# Autodesk Inventor assembly: приводной валь
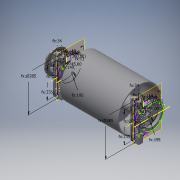
[picture p0: Inventor's stored thumbnail of the model, 180x180]
Saved by Autodesk Inventor 2018.3 (Build 223284000, 284)
## iProperties
Created: 2018-05-10
Part Number: приводной валь
Material: Типовые
Document SubType Name: Assembly
Designer: kriku
Mass: 17391.3 g
Surface Area: 20333.4 cm^2
Volume: 13778.9 cm^3
Density: 1.26217 g/cm^3
Author: kriku
## Documents named in this file (6)
- C:\Users\kriku\OneDrive\Рабочий стол\6 семестр\курсач ДМ\deadmash\Куча инви\приводной валь.iam
- C:\Users\kriku\OneDrive\Рабочий стол\6 семестр\курсач ДМ\deadmash\Куча инви\корпус подшипника1.ipt
- C:\Users\kriku\Downloads\barabashka.ipt
- C:\Users\kriku\Downloads\privodnoi_val.ipt
- C:\Users\kriku\OneDrive\Документы\Inventor\Content Center Files\R2018\ru-RU\Bearing 1000 GOST 28428-90\Подшипник 1214 ГОСТ 28428-90.ipt
- C:\Users\kriku\OneDrive\Документы\Inventor\Content Center Files\R2018\ru-RU\End Cap GOST 13219·10-81\Крышка торцовая МВ 125x70 ГОСТ 13219.10-81.ipt
## Components (7 placed, 5 different names)
1. корпус подшипника1:1 — Угол:1, Совмещение:6, Заподлицо:3
2. корпус подшипника1:2 — Угол:2, Совмещение:5, Заподлицо:2
3. barabashka:1 — Цилиндрический:1, Заподлицо:1
4. privodnoi_val:1 — Цилиндрический:1, Заподлицо:1, Совмещение:1, Совмещение:2, Совмещение:3, Совмещение:4, Совмещение:5, Совмещение:6, Совмещение:7
5. Подшипник 1000 ГОСТ 28428-90 1214:1 — Совмещение:1, Совмещение:2, Заподлицо:2
6. Подшипник 1000 ГОСТ 28428-90 1214:2 — Совмещение:3, Совмещение:4, Заподлицо:3
7. Крышка торцовая ГОСТ 13219.10-81 МВ 125x70:1 — Совмещение:7
## Relationships (13: Mate 7, Flush 3, Angle 2, CylindricalJoint 1)
- Цилиндрический:1 [CylindricalJoint]: barabashka:1 ↔ privodnoi_val:1
- Заподлицо:1 [Flush]: barabashka:1 ↔ privodnoi_val:1
- Совмещение:1 [Mate]: privodnoi_val:1 ↔ Подшипник 1000 ГОСТ 28428-90 1214:1
- Совмещение:2 [Mate]: privodnoi_val:1 ↔ Подшипник 1000 ГОСТ 28428-90 1214:1
- Совмещение:3 [Mate]: privodnoi_val:1 ↔ Подшипник 1000 ГОСТ 28428-90 1214:2
- Совмещение:4 [Mate]: privodnoi_val:1 ↔ Подшипник 1000 ГОСТ 28428-90 1214:2
- Угол:1 [Angle] (180 deg): корпус подшипника1:1
- Угол:2 [Angle] (180 deg): корпус подшипника1:2
- Совмещение:5 [Mate]: корпус подшипника1:2 ↔ privodnoi_val:1
- Заподлицо:2 [Flush] (-12 mm): корпус подшипника1:2 ↔ Подшипник 1000 ГОСТ 28428-90 1214:1
- Совмещение:6 [Mate]: корпус подшипника1:1 ↔ privodnoi_val:1
- Заподлицо:3 [Flush] (12 mm): корпус подшипника1:1 ↔ Подшипник 1000 ГОСТ 28428-90 1214:2
- Совмещение:7 [Mate]: privodnoi_val:1 ↔ Крышка торцовая ГОСТ 13219.10-81 МВ 125x70:1
